# Autodesk Inventor assembly: RobLink1
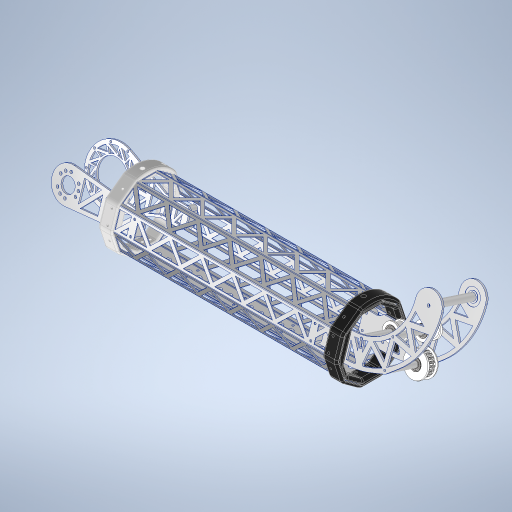
[picture p0: Inventor's stored thumbnail of the model, 512x512]
Saved by Autodesk Inventor 2024 (Build 280153000, 153)
## iProperties
Created: 2025-02-03
Part Number: RobLink1
Document SubType Name: Assembly
Designer: tanoue_kota
Mass: 521.237 g
Surface Area: 2714.1 cm^2
Volume: 281.076 cm^3
Density: 1.85444 g/cm^3
Author: tanoue_kota
## Documents named in this file (17)
- C:\Users\田之上巧太\Documents\Inventor\RobArm\rob_link1\RobLink1.iam
- C:\Users\田之上巧太\Documents\Inventor\RobArm\rob_link1\roblink1_parameter.ipt
- C:\Users\田之上巧太\Documents\Inventor\RobArm\rob_link1\link1plate1.ipt
- C:\Users\田之上巧太\Documents\Inventor\RobArm\rob_link1\link1plate2.ipt
- C:\Users\田之上巧太\Documents\Inventor\RobArm\rob_link1\link1part1.ipt
- C:\Users\田之上巧太\Documents\Inventor\RobArm\rob_link1\link1part1_MIR.ipt
- C:\Users\田之上巧太\Documents\Inventor\RobArm\rob_link1\link1part2.ipt
- C:\Users\田之上巧太\Documents\Inventor\RobArm\rob_link1\link1plate3.ipt
- C:\Users\田之上巧太\Documents\Inventor\RobArm\rob_link1\link1plate4.ipt
- C:\Users\田之上巧太\Documents\Inventor\RobArm\rob_link1\link1plate5.ipt
- C:\Users\田之上巧太\Documents\Inventor\RobArm\rob_link1\link1part3.ipt
- C:\Users\田之上巧太\Documents\Inventor\RobArm\rob_link1\link1plate5_MIR.ipt
- C:\Users\田之上巧太\Documents\Inventor\RobArm\rob_link1\link1part4.ipt
- C:\Users\田之上巧太\Documents\Inventor\RobArm\rob_link1\link1part5.ipt
- C:\Users\田之上巧太\Documents\Inventor\RobArm\rob_link1\tensioner1.ipt
- C:\Users\田之上巧太\Documents\Inventor\RobArm\BasicParts\Bearing\NMB_LF1480ZZ\LF-1480ZZ.iam
- C:\Users\田之上巧太\Documents\Inventor\RobArm\rob_link1\link1part6.ipt
## Components (29 placed, 16 different names)
1. roblink1_parameter:1
2. link1plate1:1 — 回転:1, 回転:2, 回転:5, 回転:6, 回転:7, 回転:8, 回転:9, 回転:10, 回転:11, 回転:12, 回転:13, 回転:14, 回転:15, 回転:16
3. link1plate2:1 — 回転:1, 回転:2
4. link1part1:1 — 回転:5, 回転:6, 回転:23
5. link1part1_MIR:1 — 回転:7, 回転:8, 回転:17, 回転:20
6. link1part2:1 — 回転:9, 回転:10, 回転:18
7. link1part2:2 — 回転:11, 回転:12, 回転:19
8. link1part2:3 — 回転:13, 回転:14, 回転:27
9. link1part2:4 — 回転:15, 回転:16, 回転:24
10. link1plate3:1 — 回転:17, 回転:18
11. link1plate4:1 — 回転:19, 回転:20
12. link1plate5:2 — 回転:23, 回転:24, 回転:25, 回転:28, 回転:30, 回転:31
13. link1part3:1 — 回転:25
14. link1plate5_MIR:1 — 回転:27, メイト:22, メイト:23, メイト:24
15. link1part4:1 — 回転:30, メイト:14, メイト:20
16. link1part4:2 — 回転:31, メイト:13, メイト:17
17. link1part5:1 — メイト:5, メイト:6, メイト:7, メイト:8
18. tensioner1:1 — メイト:9, メイト:10, メイト:11, メイト:12
19. link1part5:2 — メイト:1, メイト:2, メイト:3, メイト:4
20. link1part4:3 — 回転:28, メイト:15, メイト:18
21. LF-1480ZZ:1 [sub-assembly] — メイト:1, メイト:2, メイト:14, メイト:21
22. LF-1480ZZ:2 [sub-assembly] — メイト:3, メイト:4
23. LF-1480ZZ:3 [sub-assembly] — メイト:11, メイト:12
24. LF-1480ZZ:4 [sub-assembly] — メイト:9, メイト:10, メイト:13, メイト:16
25. LF-1480ZZ:5 [sub-assembly] — メイト:5, メイト:6
26. LF-1480ZZ:6 [sub-assembly] — メイト:7, メイト:8, メイト:15, メイト:19
27. link1part6:1 — メイト:18, メイト:19, メイト:24
28. link1part6:2 — メイト:20, メイト:21, メイト:23
29. link1part6:3 — メイト:16, メイト:17, メイト:22
## Relationships (49: RevoluteJoint 25, Mate 24)
- 回転:1 [RevoluteJoint]: link1plate1:1 ↔ link1plate2:1
- 回転:2 [RevoluteJoint]: link1plate1:1 ↔ link1plate2:1
- 回転:5 [RevoluteJoint]: link1plate1:1 ↔ link1part1:1
- 回転:6 [RevoluteJoint]: link1plate1:1 ↔ link1part1:1
- 回転:7 [RevoluteJoint]: link1plate1:1 ↔ link1part1_MIR:1
- 回転:8 [RevoluteJoint]: link1plate1:1 ↔ link1part1_MIR:1
- 回転:9 [RevoluteJoint]: link1plate1:1 ↔ link1part2:1
- 回転:10 [RevoluteJoint]: link1plate1:1 ↔ link1part2:1
- 回転:11 [RevoluteJoint]: link1plate1:1 ↔ link1part2:2
- 回転:12 [RevoluteJoint]: link1plate1:1 ↔ link1part2:2
- 回転:13 [RevoluteJoint]: link1plate1:1 ↔ link1part2:3
- 回転:14 [RevoluteJoint]: link1plate1:1 ↔ link1part2:3
- 回転:15 [RevoluteJoint]: link1plate1:1 ↔ link1part2:4
- 回転:16 [RevoluteJoint]: link1plate1:1 ↔ link1part2:4
- 回転:17 [RevoluteJoint]: link1part1_MIR:1 ↔ link1plate3:1
- 回転:18 [RevoluteJoint]: link1part2:1 ↔ link1plate3:1
- 回転:19 [RevoluteJoint]: link1part2:2 ↔ link1plate4:1
- 回転:20 [RevoluteJoint]: link1part1_MIR:1 ↔ link1plate4:1
- 回転:23 [RevoluteJoint]: link1part1:1 ↔ link1plate5:2
- 回転:24 [RevoluteJoint]: link1part2:4 ↔ link1plate5:2
- 回転:25 [RevoluteJoint]: link1plate5:2 ↔ link1part3:1
- 回転:27 [RevoluteJoint]: link1part2:3 ↔ link1plate5_MIR:1
- 回転:28 [RevoluteJoint]: link1plate5:2 ↔ link1part4:3
- 回転:30 [RevoluteJoint]: link1plate5:2 ↔ link1part4:1
- 回転:31 [RevoluteJoint]: link1plate5:2 ↔ link1part4:2
- メイト:1 [Mate] (0.2 mm): link1part5:2 ↔ LF-1480ZZ:1
- メイト:2 [Mate]: link1part5:2 ↔ LF-1480ZZ:1
- メイト:3 [Mate] (0.2 mm): link1part5:2 ↔ LF-1480ZZ:2
- メイト:4 [Mate]: link1part5:2 ↔ LF-1480ZZ:2
- メイト:5 [Mate] (0.2 mm): link1part5:1 ↔ LF-1480ZZ:5
- メイト:6 [Mate]: link1part5:1 ↔ LF-1480ZZ:5
- メイト:7 [Mate]: link1part5:1 ↔ LF-1480ZZ:6
- メイト:8 [Mate]: link1part5:1 ↔ LF-1480ZZ:6
- メイト:9 [Mate]: tensioner1:1 ↔ LF-1480ZZ:4
- メイト:10 [Mate]: tensioner1:1 ↔ LF-1480ZZ:4
- メイト:11 [Mate] (0.2 mm): tensioner1:1 ↔ LF-1480ZZ:3
- メイト:12 [Mate]: tensioner1:1 ↔ LF-1480ZZ:3
- メイト:13 [Mate]: link1part4:2 ↔ LF-1480ZZ:4
- メイト:14 [Mate]: link1part4:1 ↔ LF-1480ZZ:1
- メイト:15 [Mate]: link1part4:3 ↔ LF-1480ZZ:6
- メイト:16 [Mate]: LF-1480ZZ:4 ↔ link1part6:3
- メイト:17 [Mate]: link1part4:2 ↔ link1part6:3
- メイト:18 [Mate]: link1part4:3 ↔ link1part6:1
- メイト:19 [Mate]: LF-1480ZZ:6 ↔ link1part6:1
- メイト:20 [Mate]: link1part4:1 ↔ link1part6:2
- メイト:21 [Mate]: LF-1480ZZ:1 ↔ link1part6:2
- メイト:22 [Mate]: link1plate5_MIR:1 ↔ link1part6:3
- メイト:23 [Mate]: link1plate5_MIR:1 ↔ link1part6:2
- メイト:24 [Mate]: link1plate5_MIR:1 ↔ link1part6:1
